# Autodesk Inventor assembly: Rack-mount
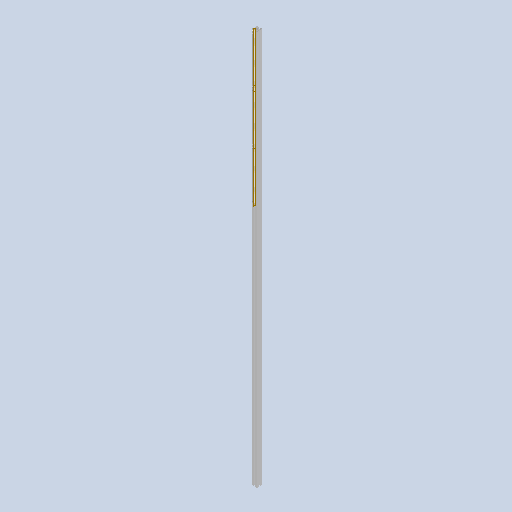
[picture p0: Inventor's stored thumbnail of the model, 512x512]
Saved by Autodesk Inventor 2023 (Build 270158000, 158)
## iProperties
Created: 2022-08-24
Part Number: Rack-mount
Document SubType Name: Assembly
Designer: matte
Author: matte
## Documents named in this file (7)
- C:\Users\matte\Documents\GitHub\MDM-CyberOrto-CAD\Rack_Pinion\Rack-mount.iam
- C:\Users\matte\Documents\GitHub\MDM-CyberOrto-CAD\Pezzi singoli\10-040.ipt
- C:\Users\matte\Documents\GitHub\MDM-CyberOrto-CAD\Rack_Pinion\Rack.ipt
- C:\Users\matte\Documents\GitHub\MDM-CyberOrto-CAD\Parker components\02-Fasteners\10-Standard T-Nuts\20-049.ipt
- C:\Users\matte\Documents\GitHub\MDM-CyberOrto-CAD\Rack_Pinion\Riduttore.ipt
- C:\Users\matte\Documents\GitHub\MDM-CyberOrto-CAD\Parker components\02-Fasteners\16-Screws\01-Metric Screws\03-Socket Head\24-320-4.ipt
- C:\Users\matte\Documents\GitHub\MDM-CyberOrto-CAD\Parker components\02-Fasteners\10-Standard T-Nuts\20-051.ipt
## Components (18 placed, 6 different names)
1. 10-040:1 — Coincidente:7, Allineato:5, Allineato:6, Coincidente:21, Coincidente:22, Coincidente:28, Angolo:1, Coincidente:31, Coincidente:32, Angolo:2
2. Rack:1 — Coincidente:2, Allineato:1, Allineato:4, Coincidente:7, Allineato:5, Allineato:6, Coincidente:18, Coincidente:20, Coincidente:33, Coincidente:34
3. Rack:2 — Coincidente:1, Coincidente:2, Allineato:1, Allineato:2, Allineato:3, Allineato:4, Coincidente:19, Coincidente:23, Coincidente:25
4. Rack:3 — Coincidente:1, Allineato:2, Allineato:3, Coincidente:24, Coincidente:29, Coincidente:30
5. 24-320-4:2 — Coincidente:10, Allineato:7, Coincidente:19
6. 24-320-4:3 — Coincidente:11, Allineato:7, Coincidente:18, Coincidente:20
7. 20-049:1 — Coincidente:3, Coincidente:4, Coincidente:5, Coincidente:6, Coincidente:21
8. Riduttore:1 — Coincidente:3, Coincidente:4, Coincidente:11
9. Riduttore:4 — Coincidente:5, Coincidente:6, Coincidente:10
10. 20-049:2 — Coincidente:22
11. Riduttore:5
12. Riduttore:6
13. 24-320-4:4 — Coincidente:23, Coincidente:25
14. 24-320-4:5 — Coincidente:24
15. 24-320-4:1 — Coincidente:26, Coincidente:29, Coincidente:30
16. 20-051:1 — Coincidente:26, Coincidente:28, Angolo:1
17. 24-320-4:6 — Coincidente:33, Coincidente:34
18. 20-051:2 — Coincidente:31, Coincidente:32, Angolo:2
## Relationships (42: Mate 32, Flush 8, Angle 2)
- Coincidente:1 [Mate]: Rack:2 ↔ Rack:3
- Coincidente:2 [Mate]: Rack:1 ↔ Rack:2
- Allineato:1 [Flush]: Rack:1 ↔ Rack:2
- Allineato:2 [Flush]: Rack:2 ↔ Rack:3
- Allineato:3 [Flush]: Rack:2 ↔ Rack:3
- Allineato:4 [Flush]: Rack:1 ↔ Rack:2
- Coincidente:3 [Mate]: 20-049:1 ↔ Riduttore:1
- Coincidente:4 [Mate]: 20-049:1 ↔ Riduttore:1
- Coincidente:5 [Mate]: 20-049:1 ↔ Riduttore:4
- Coincidente:6 [Mate]: 20-049:1 ↔ Riduttore:4
- Coincidente:7 [Mate]: 10-040:1 ↔ Rack:1
- Allineato:5 [Flush]: 10-040:1 ↔ Rack:1
- Allineato:6 [Flush] (12.5 mm): 10-040:1 ↔ Rack:1
- Coincidente:10 [Mate]: 24-320-4:2 ↔ Riduttore:4
- Coincidente:11 [Mate]: 24-320-4:3 ↔ Riduttore:1
- Allineato:7 [Flush]: 24-320-4:2 ↔ 24-320-4:3
- [Mate]: 20-049:2 ↔ Riduttore:5
- [Mate]: 20-049:2 ↔ Riduttore:5
- [Mate]: 20-049:2 ↔ Riduttore:6
- [Mate]: 20-049:2 ↔ Riduttore:6
- [Mate]: Riduttore:6 ↔ 24-320-4:4
- [Mate]: Riduttore:5 ↔ 24-320-4:5
- [Flush]: 24-320-4:4 ↔ 24-320-4:5
- Coincidente:18 [Mate]: Rack:1 ↔ 24-320-4:3
- Coincidente:19 [Mate]: Rack:2 ↔ 24-320-4:2
- Coincidente:20 [Mate]: Rack:1 ↔ 24-320-4:3
- Coincidente:21 [Mate]: 10-040:1 ↔ 20-049:1
- Coincidente:22 [Mate]: 10-040:1 ↔ 20-049:2
- Coincidente:23 [Mate]: Rack:2 ↔ 24-320-4:4
- Coincidente:24 [Mate]: Rack:3 ↔ 24-320-4:5
- Coincidente:25 [Mate]: Rack:2 ↔ 24-320-4:4
- Coincidente:26 [Mate]: 24-320-4:1 ↔ 20-051:1
- [Mate]: 24-320-4:6 ↔ 20-051:2
- Coincidente:28 [Mate]: 10-040:1 ↔ 20-051:1
- Angolo:1 [Angle] (0 deg): 10-040:1 ↔ 20-051:1
- Coincidente:29 [Mate]: Rack:3 ↔ 24-320-4:1
- Coincidente:30 [Mate]: Rack:3 ↔ 24-320-4:1
- Coincidente:31 [Mate]: 10-040:1 ↔ 20-051:2
- Coincidente:32 [Mate]: 10-040:1 ↔ 20-051:2
- Angolo:2 [Angle] (0 deg): 10-040:1 ↔ 20-051:2
- Coincidente:33 [Mate]: Rack:1 ↔ 24-320-4:6
- Coincidente:34 [Mate]: Rack:1 ↔ 24-320-4:6
## Named parameters: d28_d25 = 0 mm, d29_d26 = 0 mm, d30_d27 = 0 mm, d31_d6 = 0 mm, d32_d7 = 0 mm, d33_d8 = 0 mm, d34_d9 = 0 mm, d44_d43 = 0 mm
